# Autodesk Inventor assembly: Hand Kwik-Mount
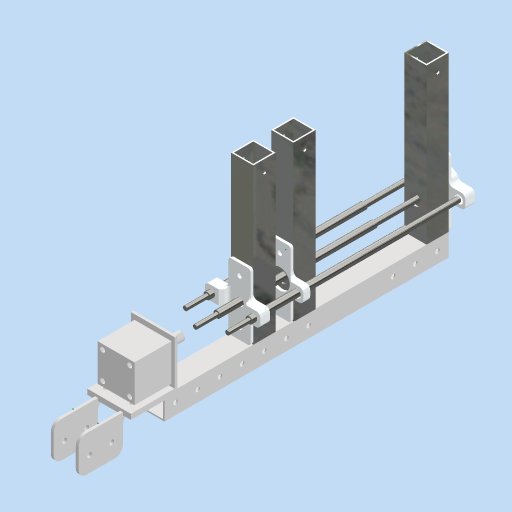
[picture p0: Inventor's stored thumbnail of the model, 512x512]
Saved by Autodesk Inventor 2024 (Build 280153000, 153)
## iProperties
Created: 2024-01-20
Part Number: Hand Kwik-Mount
Document SubType Name: Assembly
Designer: aidan
Author: aidan
## Documents named in this file (13)
- C:\Users\megan\OneDrive\Documents\GitHub\BehrendURCMechanical\CAD\Chassis V3\Robotic Claw\CH - Hand W Standard Gussets.iam
- C:\Users\aidan\OneDrive\Documents\Inventor\Content Center Files\am-4158 1IN Tee Gusset.ipt
- C:\Users\aidan\OneDrive\Documents\Inventor\Content Center Files\am-3860 90 Gusset REV2.ipt
- C:\Users\megan\OneDrive\Documents\GitHub\BehrendURCMechanical\CAD\Chassis V3\Robotic Claw\Tube Finger.ipt
- C:\Users\megan\OneDrive\Documents\GitHub\BehrendURCMechanical\CAD\Chassis V3\Robotic Claw\Lead Nut Holder Mk2.ipt
- C:\Users\megan\OneDrive\Documents\GitHub\BehrendURCMechanical\CAD\Chassis V3\Robotic Claw\Guide Rod Holder.ipt
- C:\Users\megan\OneDrive\Documents\GitHub\BehrendURCMechanical\CAD\Chassis V3\Robotic Claw\Finger Base.ipt
- C:\Users\megan\OneDrive\Documents\GitHub\BehrendURCMechanical\CAD\Chassis V3\Robotic Claw\Lead_Shaft.ipt
- C:\Users\megan\OneDrive\Documents\GitHub\BehrendURCMechanical\CAD\Chassis V3\Robotic Claw\Nema 3 Mounting.ipt
- C:\Users\megan\OneDrive\Documents\GitHub\BehrendURCMechanical\CAD\Chassis V3\Robotic Claw\Nema 17.ipt
- C:\Users\megan\OneDrive\Documents\GitHub\BehrendURCMechanical\CAD\Chassis V3\Robotic Claw\Motor Mount.ipt
- C:\Users\megan\OneDrive\Documents\GitHub\BehrendURCMechanical\CAD\Chassis V3\Robotic Claw\Bearing Holder.ipt
- C:\Users\megan\OneDrive\Documents\GitHub\BehrendURCMechanical\CAD\Chassis V3\Robotic Claw\Shaft Adapter.ipt
## Components (18 placed, 12 different names)
1. am-3860 90 Gusset REV2:1
2. am-3860 90 Gusset REV2:2 — Rotational:4
3. Tube Finger:1 — Mate:1, Rotational:12
4. Tube Finger:2 — Mate:1
5. Lead Nut Holder Mk2:1
6. Tube Finger:3 — Rotational:7
7. Finger Base:1 — Rotational:4, Rotational:5, Rotational:6, Rotational:14
8. am-4158 1IN Tee Gusset:1 — Rotational:6
9. am-4158 1IN Tee Gusset:2 — Rotational:5
10. Guide Rod Holder:2 — Rotational:7, Rotational:8, Rotational:9, Rotational:10
11. Lead_Shaft:1 — Rotational:10
12. Lead_Shaft:2 — Rotational:9
13. Lead_Shaft:3 — Rotational:8
14. Nema 3 Mounting:1 — Rotational:15
15. Nema 17:1 — Rotational:16
16. Motor Mount:1 — Rotational:14, Rotational:15
17. Bearing Holder:1 — Rotational:12
18. Shaft Adapter:1 — Rotational:16
## Relationships (12: RevoluteJoint 11, Mate 1)
- Mate:1 (127 mm): Tube Finger:1 ↔ Tube Finger:2
- Rotational:4 [RevoluteJoint]: am-3860 90 Gusset REV2:2 ↔ Finger Base:1
- Rotational:5 [RevoluteJoint]: Finger Base:1 ↔ am-4158 1IN Tee Gusset:2
- Rotational:6 [RevoluteJoint]: Finger Base:1 ↔ am-4158 1IN Tee Gusset:1
- Rotational:7 [RevoluteJoint]: Tube Finger:3 ↔ Guide Rod Holder:2
- Rotational:8 [RevoluteJoint] (-38.1 mm): Guide Rod Holder:2 ↔ Lead_Shaft:3
- Rotational:9 [RevoluteJoint] (-50.8 mm): Guide Rod Holder:2 ↔ Lead_Shaft:2
- Rotational:10 [RevoluteJoint] (-38.1 mm): Guide Rod Holder:2 ↔ Lead_Shaft:1
- Rotational:12 [RevoluteJoint]: Tube Finger:1 ↔ Bearing Holder:1
- Rotational:14 [RevoluteJoint]: Finger Base:1 ↔ Motor Mount:1
- Rotational:15 [RevoluteJoint]: Nema 3 Mounting:1 ↔ Motor Mount:1
- Rotational:16 [RevoluteJoint] (-6.35 mm): Nema 17:1 ↔ Shaft Adapter:1
